# Autodesk Inventor assembly: Assembly3
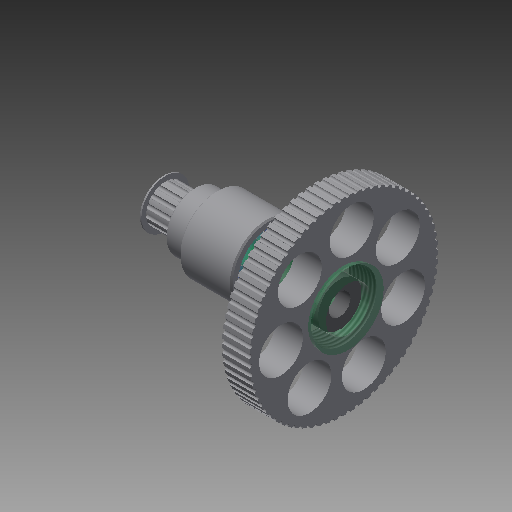
[picture p0: Inventor's stored thumbnail of the model, 512x512]
Saved by Autodesk Inventor 2018.1 (Build 221171000, 171)
## iProperties
Created: 2022-06-29
Part Number: Assembly3
Document SubType Name: Assembly
Designer: Bureau
Author: Bureau
## Documents named in this file (3)
- C:\Users\mouta\GoogleDrive\Manu\USINAGE\MoteurVelo\Arbre secondaire\Assembly3.iam
- C:\Users\mouta\GoogleDrive\Manu\USINAGE\MoteurVelo\Arbre secondaire\Assembly1.iam
- C:\Users\mouta\GoogleDrive\Manu\USINAGE\MoteurVelo\Arbre secondaire\Assembly2.iam
## Components (2 placed, 2 different names)
1. Assembly1:1 [sub-assembly] — Mate:1, Mate:2
2. Assembly2:1 [sub-assembly] — Mate:1, Mate:2
## Relationships (2: Mate 2)
- Mate:1: Assembly1:1 ↔ Assembly2:1
- Mate:2: Assembly1:1 ↔ Assembly2:1
